# Autodesk Inventor assembly: Ensamble NotAFarmBot2
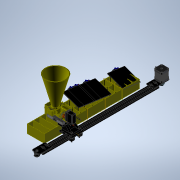
[picture p0: Inventor's stored thumbnail of the model, 180x180]
Saved by Autodesk Inventor 2020.3 (Build 243373000, 373)
## iProperties
Created: 2020-07-22
Part Number: Ensamble NotAFarmBot2
Document SubType Name: Assembly
Designer: juanp
Mass: 1932.13 g
Surface Area: 7509.2 cm^2
Volume: 1044.57 cm^3
Density: 1.84968 g/cm^3
Author: juanp
## Documents named in this file (23)
- C:\Users\juanp\Desktop\Robocol\Diseño EVA\Ensamble EVA.iam
- C:\Users\juanp\Desktop\Robocol\Diseño EVA\Actuador Lineal\VSLOT 2020 Extrusion.ipt
- C:\Users\juanp\Desktop\Robocol\Diseño EVA\Actuador Lineal\VSLOT Complementarios\Double Tee Nut.ipt
- C:\Users\juanp\Desktop\Robocol\Diseño EVA\Actuador Lineal\GT2_30T_5_6.ipt
- C:\Users\juanp\Desktop\Robocol\Diseño EVA\Actuador Lineal\Idler Pulley Plate.ipt
- C:\Users\juanp\Desktop\Robocol\Diseño EVA\Actuador Lineal\Motor Mount Plate Nema 17.ipt
- C:\Users\juanp\Desktop\Robocol\Diseño EVA\Actuador Lineal\M1173041- NEMA 17.ipt
- C:\Users\juanp\Desktop\Robocol\Diseño EVA\Actuador Lineal\Placas deslizantes\20mm Gantry Set.iam
- C:\Users\juanp\Desktop\Robocol\Diseño EVA\Actuador Lineal\VSLOT Complementarios\3mm Spacer.ipt
- C:\Users\juanp\Desktop\Robocol\Diseño EVA\Actuador Lineal\VSLOT Complementarios\M5x25 low profile screw.ipt
- C:\Users\juanp\Desktop\Robocol\Diseño EVA\Actuador Lineal\VSLOT Complementarios\Ball Bearing 625 2RS 5x16x5.ipt
- C:\Users\juanp\Desktop\Robocol\Diseño EVA\Actuador Lineal\VSLOT Complementarios\1mm 5mm shim.ipt
- C:\Users\juanp\Desktop\Robocol\Diseño EVA\Actuador Lineal\VSLOT Complementarios\Nylon Spacer 1_8th.ipt
- C:\Users\juanp\Desktop\Robocol\Diseño EVA\Actuador Lineal\VSLOT Complementarios\idler pulley.ipt
- C:\Users\juanp\Desktop\Robocol\Diseño EVA\Actuador Lineal\Placas deslizantes\M5 Nylock.ipt
- C:\Users\juanp\Desktop\Robocol\Diseño EVA\Actuador Lineal\VSLOT Complementarios\M5x8 low profile screw.ipt
- C:\Users\juanp\Documents\Inventor\Content Center Files\R2020\en-US\ANSI B18.3.4M(1)\ANSI B18.3.4M - M3 x 0.5 x 8(2).ipt
- C:\Users\juanp\Desktop\Robocol\Diseño EVA\Dispensador\Ensamble Dispensador V2.iam
- C:\Users\juanp\Desktop\Robocol\Diseño EVA\Contenedores\Contenedor3.ipt
- C:\Users\juanp\Desktop\Robocol\Diseño EVA\CADs Sensores\Sensor gas MQX\MQ2 Gas Sensor.ipt
- C:\Users\juanp\Documents\Inventor\Content Center Files\R2020\en-US\ANSI B18.2.3.5M\ANSI B18.2.3.5M - M5 x 0.8 x 40.ipt
- C:\Users\juanp\Desktop\Robocol\Diseño EVA\Contenedores\TapasContenedor.ipt
- C:\Users\juanp\Desktop\Robocol\Diseño EVA\Contenedores\Servo SG90\SG90 - Micro Servo 9g - Tower Pro.1.ipt
## Components (41 placed, 22 different names)
1. VSLOT 2020 Extrusion:1 — Mate:85, Mate:86, Mate:87, Mate:88, Angle:16, Mate:98, Mate:99, Angle:18, Mate:100, Mate:101, Angle:23, Mate:185, Angle:24, Tangent:1, Tangent:2, Flush:1, Angle:25, Tangent:3, Tangent:4, Flush:3, Mate:196, Mate:197, Flush:6
2. Double Tee Nut:1 — Mate:98, Mate:99, Angle:18, Mate:100, Mate:106
3. Double Tee Nut:2 — Mate:85, Mate:86, Mate:87, Mate:93, Angle:16, Mate:94
4. GT2_30T_5_6:2 — Mate:35, Mate:107
5. Idler Pulley Plate:1 — Mate:88, Mate:89, Mate:90, Mate:91, Mate:92, Mate:95, Mate:96, Mate:97, Angle:17
6. Motor Mount Plate Nema 17:1 — Mate:12, Mate:13, Angle:4, Mate:42, Mate:43, Mate:52, Mate:53, Mate:54, Mate:55, Mate:101, Mate:102, Mate:103, Mate:104, Mate:105, Angle:24
7. M1173041- NEMA 17:1 — Mate:12, Mate:13, Angle:4, Mate:48, Mate:49, Mate:50, Mate:51, Mate:107
8. 20mm Gantry Set:1 [sub-assembly] — Angle:23, Mate:186, Tangent:1, Tangent:2, Tangent:3, Tangent:4, Mate:189, Mate:191, Mate:198, Mate:199, Mate:200
9. M5x25 low profile screw:1 — Mate:27, Mate:28, Mate:29, Mate:31, Mate:46, Mate:96
10. Ball Bearing 625 2RS 5x16x5:1 — Mate:22, Mate:23, Mate:24, Mate:26, Mate:32
11. Ball Bearing 625 2RS 5x16x5:2 — Mate:21, Mate:25, Mate:28
12. 1mm 5mm shim:1 — Mate:29, Mate:47, Mate:97
13. Nylon Spacer 1_8th:1 — Mate:23, Mate:24, Mate:25
14. idler pulley:1 — Mate:21, Mate:22, Mate:26, Mate:27, Mate:35
15. 3mm Spacer:1 — Mate:31, Mate:32, Mate:95
16. M5x8 low profile screw:1 — Mate:42, Mate:102, Mate:104
17. M5x8 low profile screw:2 — Mate:43, Mate:103, Mate:105, Mate:106
18. M5x8 low profile screw:3 — Mate:90, Mate:92, Mate:94
19. M5x8 low profile screw:4 — Mate:89, Mate:91, Mate:93
20. M5 Nylock:1 — Mate:46, Mate:47, Angle:17
21. Broached Hexagon Socket Button Head Cap Screw - Metric M3 x 0.5 x 8:1 — Mate:50, Mate:54
22. Broached Hexagon Socket Button Head Cap Screw - Metric M3 x 0.5 x 8:2 — Mate:51, Mate:55
23. Broached Hexagon Socket Button Head Cap Screw - Metric M3 x 0.5 x 8:3 — Mate:49, Mate:52
24. Broached Hexagon Socket Button Head Cap Screw - Metric M3 x 0.5 x 8:4 — Mate:48, Mate:53
25. Ensamble Dispensador V2:1 [sub-assembly] — Mate:186, Mate:190, Mate:191, Mate:201
26. Contenedor3:1 — Flush:1, Angle:25, Mate:189, Mate:190, Angle:26, Flush:6, Mate:203, Mate:204, Mate:205, Mate:208, Mate:209, Mate:210, Mate:211, Mate:212
27. MQ2 Gas Sensor:1 — Angle:26
28. Hex Bolt - Metric M5 x 0.8 x 40:3 — Flush:4, Mate:198
29. Hex Bolt - Metric M5 x 0.8 x 40:2 — Flush:4, Flush:5, Mate:199, Mate:201
30. Hex Bolt - Metric M5 x 0.8 x 40:1 — Flush:5, Mate:200
31. MQ2 Gas Sensor:2
32. MQ2 Gas Sensor:3
33. MQ2 Gas Sensor:4
34. TapasContenedor:1 — Mate:206, Mate:207, Flush:13
35. SG90 - Micro Servo 9g - Tower Pro.1:2 — Mate:203, Mate:204, Mate:205, Mate:206, Mate:207
36. SG90 - Micro Servo 9g - Tower Pro.1:3 — Mate:208, Flush:7, Flush:10, Mate:211, Mate:212, Mate:215
37. SG90 - Micro Servo 9g - Tower Pro.1:4 — Mate:209, Flush:7, Flush:8, Flush:9, Flush:10, Mate:216
38. SG90 - Micro Servo 9g - Tower Pro.1:5 — Mate:210, Flush:8, Flush:9, Mate:217, Mate:218
39. TapasContenedor:2 — Mate:213, Mate:215, Flush:12, Flush:13
40. TapasContenedor:3 — Mate:213, Mate:214, Mate:216, Flush:11, Flush:12
41. TapasContenedor:4 — Mate:214, Mate:217, Mate:218, Flush:11
## Relationships (100: Mate 76, Flush 12, Angle 8, Tangent 4)
- Mate:12: Motor Mount Plate Nema 17:1 ↔ M1173041- NEMA 17:1
- Mate:13: Motor Mount Plate Nema 17:1 ↔ M1173041- NEMA 17:1
- Angle:4 (0 deg): Motor Mount Plate Nema 17:1 ↔ M1173041- NEMA 17:1
- Mate:21: Ball Bearing 625 2RS 5x16x5:2 ↔ idler pulley:1
- Mate:22: Ball Bearing 625 2RS 5x16x5:1 ↔ idler pulley:1
- Mate:23: Ball Bearing 625 2RS 5x16x5:1 ↔ Nylon Spacer 1_8th:1
- Mate:24: Ball Bearing 625 2RS 5x16x5:1 ↔ Nylon Spacer 1_8th:1
- Mate:25: Ball Bearing 625 2RS 5x16x5:2 ↔ Nylon Spacer 1_8th:1
- Mate:26: Ball Bearing 625 2RS 5x16x5:1 ↔ idler pulley:1
- Mate:27: M5x25 low profile screw:1 ↔ idler pulley:1
- Mate:28: M5x25 low profile screw:1 ↔ Ball Bearing 625 2RS 5x16x5:2
- Mate:29: M5x25 low profile screw:1 ↔ 1mm 5mm shim:1
- Mate:31: M5x25 low profile screw:1 ↔ 3mm Spacer:1
- Mate:32: Ball Bearing 625 2RS 5x16x5:1 ↔ 3mm Spacer:1
- Mate:35: GT2_30T_5_6:2 ↔ idler pulley:1
- Mate:42: Motor Mount Plate Nema 17:1 ↔ M5x8 low profile screw:1
- Mate:43: Motor Mount Plate Nema 17:1 ↔ M5x8 low profile screw:2
- Mate:46: M5x25 low profile screw:1 ↔ M5 Nylock:1
- Mate:47: 1mm 5mm shim:1 ↔ M5 Nylock:1
- Mate:48: M1173041- NEMA 17:1 ↔ Broached Hexagon Socket Button Head Cap Screw - Metric M3 x 0.5 x 8:4
- Mate:49: M1173041- NEMA 17:1 ↔ Broached Hexagon Socket Button Head Cap Screw - Metric M3 x 0.5 x 8:3
- Mate:50: M1173041- NEMA 17:1 ↔ Broached Hexagon Socket Button Head Cap Screw - Metric M3 x 0.5 x 8:1
- Mate:51: M1173041- NEMA 17:1 ↔ Broached Hexagon Socket Button Head Cap Screw - Metric M3 x 0.5 x 8:2
- Mate:52: Motor Mount Plate Nema 17:1 ↔ Broached Hexagon Socket Button Head Cap Screw - Metric M3 x 0.5 x 8:3
- Mate:53: Motor Mount Plate Nema 17:1 ↔ Broached Hexagon Socket Button Head Cap Screw - Metric M3 x 0.5 x 8:4
- Mate:54: Motor Mount Plate Nema 17:1 ↔ Broached Hexagon Socket Button Head Cap Screw - Metric M3 x 0.5 x 8:1
- Mate:55: Motor Mount Plate Nema 17:1 ↔ Broached Hexagon Socket Button Head Cap Screw - Metric M3 x 0.5 x 8:2
- Mate:85: VSLOT 2020 Extrusion:1 ↔ Double Tee Nut:2
- Mate:86 (-10 mm): VSLOT 2020 Extrusion:1 ↔ Double Tee Nut:2
- Mate:87: VSLOT 2020 Extrusion:1 ↔ Double Tee Nut:2
- Mate:88: VSLOT 2020 Extrusion:1 ↔ Idler Pulley Plate:1
- Mate:89: Idler Pulley Plate:1 ↔ M5x8 low profile screw:4
- Mate:90: Idler Pulley Plate:1 ↔ M5x8 low profile screw:3
- Mate:91: Idler Pulley Plate:1 ↔ M5x8 low profile screw:4
- Mate:92: Idler Pulley Plate:1 ↔ M5x8 low profile screw:3
- Mate:93: Double Tee Nut:2 ↔ M5x8 low profile screw:4
- Angle:16 (180 deg): VSLOT 2020 Extrusion:1 ↔ Double Tee Nut:2
- Mate:94: Double Tee Nut:2 ↔ M5x8 low profile screw:3
- Mate:95: Idler Pulley Plate:1 ↔ 3mm Spacer:1
- Mate:96: Idler Pulley Plate:1 ↔ M5x25 low profile screw:1
- Mate:97: Idler Pulley Plate:1 ↔ 1mm 5mm shim:1
- Angle:17 (0 deg): Idler Pulley Plate:1 ↔ M5 Nylock:1
- Mate:98: VSLOT 2020 Extrusion:1 ↔ Double Tee Nut:1
- Mate:99: VSLOT 2020 Extrusion:1 ↔ Double Tee Nut:1
- Angle:18 (0 deg): VSLOT 2020 Extrusion:1 ↔ Double Tee Nut:1
- Mate:100 (-10 mm): VSLOT 2020 Extrusion:1 ↔ Double Tee Nut:1
- Mate:101: VSLOT 2020 Extrusion:1 ↔ Motor Mount Plate Nema 17:1
- Mate:102: Motor Mount Plate Nema 17:1 ↔ M5x8 low profile screw:1
- Mate:103: Motor Mount Plate Nema 17:1 ↔ M5x8 low profile screw:2
- Mate:104: Motor Mount Plate Nema 17:1 ↔ M5x8 low profile screw:1
- Mate:105: Motor Mount Plate Nema 17:1 ↔ M5x8 low profile screw:2
- Mate:106: Double Tee Nut:1 ↔ M5x8 low profile screw:2
- Mate:107: GT2_30T_5_6:2 ↔ M1173041- NEMA 17:1
- Angle:23 (0 deg): VSLOT 2020 Extrusion:1 ↔ 20mm Gantry Set:1
- Mate:185: VSLOT 2020 Extrusion:1
- Angle:24 (0 deg): VSLOT 2020 Extrusion:1 ↔ Motor Mount Plate Nema 17:1
- Mate:186: 20mm Gantry Set:1 ↔ Ensamble Dispensador V2:1
- Tangent:1: VSLOT 2020 Extrusion:1 ↔ 20mm Gantry Set:1
- Tangent:2: VSLOT 2020 Extrusion:1 ↔ 20mm Gantry Set:1
- Flush:1: VSLOT 2020 Extrusion:1 ↔ Contenedor3:1
- Angle:25 (0 deg): VSLOT 2020 Extrusion:1 ↔ Contenedor3:1
- Tangent:3: VSLOT 2020 Extrusion:1 ↔ 20mm Gantry Set:1
- Tangent:4: VSLOT 2020 Extrusion:1 ↔ 20mm Gantry Set:1
- Mate:189 (5 mm): 20mm Gantry Set:1 ↔ Contenedor3:1
- Mate:190: Ensamble Dispensador V2:1 ↔ Contenedor3:1
- Mate:191: 20mm Gantry Set:1 ↔ Ensamble Dispensador V2:1
- Flush:3: VSLOT 2020 Extrusion:1
- Mate:196: VSLOT 2020 Extrusion:1
- Mate:197: VSLOT 2020 Extrusion:1
- Flush:4: Hex Bolt - Metric M5 x 0.8 x 40:3 ↔ Hex Bolt - Metric M5 x 0.8 x 40:2
- Flush:5: Hex Bolt - Metric M5 x 0.8 x 40:2 ↔ Hex Bolt - Metric M5 x 0.8 x 40:1
- Mate:198: 20mm Gantry Set:1 ↔ Hex Bolt - Metric M5 x 0.8 x 40:3
- Mate:199: 20mm Gantry Set:1 ↔ Hex Bolt - Metric M5 x 0.8 x 40:2
- Mate:200: 20mm Gantry Set:1 ↔ Hex Bolt - Metric M5 x 0.8 x 40:1
- Mate:201: Ensamble Dispensador V2:1 ↔ Hex Bolt - Metric M5 x 0.8 x 40:2
- Angle:26 (0 deg): Contenedor3:1 ↔ MQ2 Gas Sensor:1
- Flush:6: VSLOT 2020 Extrusion:1 ↔ Contenedor3:1
- Mate:203: Contenedor3:1 ↔ SG90 - Micro Servo 9g - Tower Pro.1:2
- Mate:204: Contenedor3:1 ↔ SG90 - Micro Servo 9g - Tower Pro.1:2
- Mate:205: Contenedor3:1 ↔ SG90 - Micro Servo 9g - Tower Pro.1:2
- Mate:206: TapasContenedor:1 ↔ SG90 - Micro Servo 9g - Tower Pro.1:2
- Mate:207: TapasContenedor:1 ↔ SG90 - Micro Servo 9g - Tower Pro.1:2
- Mate:208: Contenedor3:1 ↔ SG90 - Micro Servo 9g - Tower Pro.1:3
- Mate:209: Contenedor3:1 ↔ SG90 - Micro Servo 9g - Tower Pro.1:4
- Mate:210: Contenedor3:1 ↔ SG90 - Micro Servo 9g - Tower Pro.1:5
- Flush:7: SG90 - Micro Servo 9g - Tower Pro.1:3 ↔ SG90 - Micro Servo 9g - Tower Pro.1:4
- Flush:8: SG90 - Micro Servo 9g - Tower Pro.1:4 ↔ SG90 - Micro Servo 9g - Tower Pro.1:5
- Flush:9: SG90 - Micro Servo 9g - Tower Pro.1:4 ↔ SG90 - Micro Servo 9g - Tower Pro.1:5
- Flush:10: SG90 - Micro Servo 9g - Tower Pro.1:3 ↔ SG90 - Micro Servo 9g - Tower Pro.1:4
- Mate:211: Contenedor3:1 ↔ SG90 - Micro Servo 9g - Tower Pro.1:3
- Mate:212: Contenedor3:1 ↔ SG90 - Micro Servo 9g - Tower Pro.1:3
- Mate:213: TapasContenedor:2 ↔ TapasContenedor:3
- Mate:214: TapasContenedor:3 ↔ TapasContenedor:4
- Mate:215: SG90 - Micro Servo 9g - Tower Pro.1:3 ↔ TapasContenedor:2
- Mate:216: SG90 - Micro Servo 9g - Tower Pro.1:4 ↔ TapasContenedor:3
- Mate:217: SG90 - Micro Servo 9g - Tower Pro.1:5 ↔ TapasContenedor:4
- Mate:218: SG90 - Micro Servo 9g - Tower Pro.1:5 ↔ TapasContenedor:4
- Flush:11: TapasContenedor:3 ↔ TapasContenedor:4
- Flush:12: TapasContenedor:2 ↔ TapasContenedor:3
- Flush:13: TapasContenedor:1 ↔ TapasContenedor:2
